# Autodesk Inventor assembly: SpeleoFox
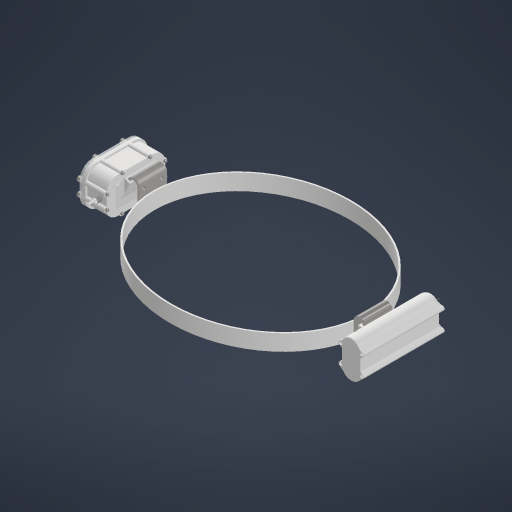
[picture p0: Inventor's stored thumbnail of the model, 512x512]
Saved by Autodesk Inventor 2024 (Build 280153000, 153)
## iProperties
Created: 2026-08-20
Part Number: SpeleoFox
Document SubType Name: Assembly
Designer: schar
Author: schar
## Documents named in this file (4)
- C:\Users\schar\Projects\SpeleoFox\cad\SpeleoFox.iam
- C:\Users\schar\Projects\SpeleoFox\cad\speleofox_parts\back_assembly.iam
- C:\Users\schar\Projects\SpeleoFox\cad\speleofox_parts\SpeleoFox_front.iam
- C:\Users\schar\Projects\SpeleoFox\cad\speleofox_parts\mounting_ring.ipt
## Components (3 placed, 3 different names)
1. back_assembly:1 [sub-assembly] — Flush:1, Mate:1, Flush:3
2. SpeleoFox_front:1 [sub-assembly] — Flush:2, Mate:1, Flush:3
3. mounting_ring:1 — Flush:1, Flush:2
## Relationships (4: Flush 3, Mate 1)
- Flush:1: back_assembly:1 ↔ mounting_ring:1
- Flush:2: SpeleoFox_front:1 ↔ mounting_ring:1
- Mate:1 (240 mm): back_assembly:1 ↔ SpeleoFox_front:1
- Flush:3: back_assembly:1 ↔ SpeleoFox_front:1
